# Autodesk Inventor assembly: main climber
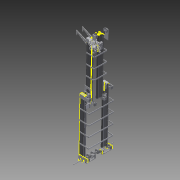
[picture p0: Inventor's stored thumbnail of the model, 180x180]
Saved by Autodesk Inventor 2013 (Build 170138000, 138)
## iProperties
Created: 2013-01-25
Part Number: main climber
Document SubType Name: Assembly
Designer: Arpan
Mass: 8312.08 g
Surface Area: 14640.7 cm^2
Volume: 3315.49 cm^3
Density: 2.50704 g/cm^3
Author: Arpan
## Documents named in this file (10)
- C:\Users\Arpan\Documents\GitHub\frc2013CAD\Cimber actual\main climber.iam
- C:\Users\Arpan\Documents\GitHub\frc2013CAD\Cimber actual\14 inch shaft.ipt
- C:\Users\Arpan\Documents\GitHub\frc2013CAD\Cimber actual\Inner rails.iam
- C:\Users\Arpan\Documents\GitHub\frc2013CAD\Cimber actual\outer rails.iam
- C:\Users\Arpan\Documents\GitHub\frc2013CAD\Cimber actual\small pulley assembly.iam
- C:\Users\Arpan\Documents\GitHub\frc2013CAD\Cimber actual\endstop 5.ipt
- C:\Users\Arpan\Documents\GitHub\frc2013CAD\Cimber actual\rough pulley.ipt
- C:\Users\Arpan\Documents\GitHub\frc2013CAD\Cimber actual\bottom pulley mount.ipt
- C:\Users\Arpan\Documents\GitHub\frc2013CAD\Cimber actual\Sideways pulley mount.iam
- C:\Users\Arpan\Documents\GitHub\frc2013CAD\Cimber actual\Sideways pulley mount 2.iam
## Components (20 placed, 9 different names)
1. Inner rails:1 [sub-assembly] — Mate:1, Angle:1, Flush:1, Mate:3, Mate:5, Flush:5, Flush:6, Mate:6, Mate:7, Mate:14, Mate:15, Mate:16, Mate:17, Mate:18, Mate:19, Mate:26, Mate:27, Flush:7
2. outer rails:1 [sub-assembly] — Mate:1, Mate:2, Angle:1, Flush:1, Flush:4, Mate:8, Mate:9, Mate:10, Mate:11, Mate:20, Mate:21, Mate:22, Mate:23, Mate:24, Mate:25, Mate:28, Mate:29, Mate:36, Flush:9, Mate:37, Flush:10, Flush:11, Mate:38, Mate:39, Mate:47, Mate:48
3. 14 inch shaft:1 — Mate:2, Flush:4, Mate:30, Mate:31, Mate:32
4. small pulley assembly:1 [sub-assembly] — Mate:5, Flush:5, Flush:6
5. small pulley assembly:2 [sub-assembly] — Mate:3, Mate:6, Mate:7
6. small pulley assembly:3 [sub-assembly] — Mate:8, Mate:9, Mate:10
7. small pulley assembly:4 [sub-assembly] — Mate:11, Mate:47, Mate:48
8. small pulley assembly:5 [sub-assembly] — Mate:17, Mate:18, Mate:19
9. small pulley assembly:6 [sub-assembly] — Mate:14, Mate:15, Mate:16
10. small pulley assembly:8 [sub-assembly] — Mate:23, Mate:24, Mate:25
11. small pulley assembly:9 [sub-assembly] — Mate:20, Mate:21, Mate:22
12. endstop 5:1 — Mate:28, Mate:29
13. endstop 5:2 — Mate:26, Mate:27
14. rough pulley:1 — Mate:31, Flush:8
15. rough pulley:2 — Mate:30, Mate:33
16. rough pulley:3 — Mate:32, Mate:35
17. bottom pulley mount:1 — Mate:37, Flush:10, Flush:11, Flush:12, Mate:40, Mate:41
18. bottom pulley mount:2 — Mate:36, Flush:9, Mate:38, Mate:39, Mate:45, Mate:46
19. Sideways pulley mount:1 [sub-assembly] — Flush:12, Mate:40, Mate:41, Flush:13
20. Sideways pulley mount 2:1 [sub-assembly] — Mate:45, Mate:46, Flush:13
## Relationships (53: Mate 41, Flush 11, Angle 1)
- Mate:1: Inner rails:1 ↔ outer rails:1
- Mate:2: outer rails:1 ↔ 14 inch shaft:1
- Angle:1 (180 deg): Inner rails:1 ↔ outer rails:1
- Flush:1 (508 mm): Inner rails:1 ↔ outer rails:1
- Flush:4 (-82.8929 mm): outer rails:1 ↔ 14 inch shaft:1
- Mate:3: Inner rails:1 ↔ small pulley assembly:2
- Mate:5: Inner rails:1 ↔ small pulley assembly:1
- Flush:5: Inner rails:1 ↔ small pulley assembly:1
- Flush:6: Inner rails:1 ↔ small pulley assembly:1
- Mate:6: Inner rails:1 ↔ small pulley assembly:2
- Mate:7: Inner rails:1 ↔ small pulley assembly:2
- Mate:8: outer rails:1 ↔ small pulley assembly:3
- Mate:9: outer rails:1 ↔ small pulley assembly:3
- Mate:10: outer rails:1 ↔ small pulley assembly:3
- Mate:11: outer rails:1 ↔ small pulley assembly:4
- Mate:14: Inner rails:1 ↔ small pulley assembly:6
- Mate:15: Inner rails:1 ↔ small pulley assembly:6
- Mate:16: Inner rails:1 ↔ small pulley assembly:6
- Mate:17: Inner rails:1 ↔ small pulley assembly:5
- Mate:18: Inner rails:1 ↔ small pulley assembly:5
- Mate:19: Inner rails:1 ↔ small pulley assembly:5
- Mate:20: outer rails:1 ↔ small pulley assembly:9
- Mate:21: outer rails:1 ↔ small pulley assembly:9
- Mate:22: outer rails:1 ↔ small pulley assembly:9
- Mate:23: outer rails:1 ↔ small pulley assembly:8
- Mate:24: outer rails:1 ↔ small pulley assembly:8
- Mate:25: outer rails:1 ↔ small pulley assembly:8
- Mate:26: Inner rails:1 ↔ endstop 5:2
- Mate:27: Inner rails:1 ↔ endstop 5:2
- Mate:28: outer rails:1 ↔ endstop 5:1
- Mate:29: outer rails:1 ↔ endstop 5:1
- Mate:30: 14 inch shaft:1 ↔ rough pulley:2
- Mate:31: 14 inch shaft:1 ↔ rough pulley:1
- Mate:32: 14 inch shaft:1 ↔ rough pulley:3
- Flush:7 (-6.35 mm): Inner rails:1
- Mate:33 (-10.3188 mm): rough pulley:2
- Mate:35 (-61.1188 mm): rough pulley:3
- Flush:8 (-61.1188 mm): rough pulley:1
- Mate:36: outer rails:1 ↔ bottom pulley mount:2
- Flush:9: outer rails:1 ↔ bottom pulley mount:2
- Mate:37: outer rails:1 ↔ bottom pulley mount:1
- Flush:10: outer rails:1 ↔ bottom pulley mount:1
- Flush:11 (12.192 mm): outer rails:1 ↔ bottom pulley mount:1
- Mate:38: outer rails:1 ↔ bottom pulley mount:2
- Mate:39: outer rails:1 ↔ bottom pulley mount:2
- Flush:12 (1.5875 mm): bottom pulley mount:1 ↔ Sideways pulley mount:1
- Mate:40: bottom pulley mount:1 ↔ Sideways pulley mount:1
- Mate:41: bottom pulley mount:1 ↔ Sideways pulley mount:1
- Mate:45: bottom pulley mount:2 ↔ Sideways pulley mount 2:1
- Mate:46: bottom pulley mount:2 ↔ Sideways pulley mount 2:1
- Flush:13: Sideways pulley mount:1 ↔ Sideways pulley mount 2:1
- Mate:47: outer rails:1 ↔ small pulley assembly:4
- Mate:48: outer rails:1 ↔ small pulley assembly:4
